# Autodesk Inventor assembly: P1704_E2
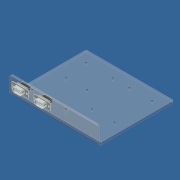
[picture p0: Inventor's stored thumbnail of the model, 180x180]
Saved by Autodesk Inventor 2015 SP2 (Build 190223200, 223)
## iProperties
Created: 2018-05-15
Part Number: P1704_E2
Project: Manette arcade
Description: Console
Document SubType Name: Assembly
Designer: Alexandre.PICOTTE
Author: Alexandre.PICOTTE
## Documents named in this file (3)
- C:\Users\Alexandre.PICOTTE\Documents\P1704_Manettes\06_Dessins\Manette_arcade\P1704_E2.iam
- C:\Users\Alexandre.PICOTTE\Documents\P1704_Manettes\06_Dessins\Manette_arcade\P1704_007.ipt
- C:\Users\Alexandre.PICOTTE\Documents\Inventor\Content Center Files\R2015\fr-FR\D-Sub Male Crimp\D-Sub Male Crimp 9CKT.ipt
## Components (3 placed, 2 different names)
1. P1704_007:1 — Placage:1, Placage:2, Placage:3, Placage:4, Angle:1, Angle:2
2. Sertissage mâle D-Sub D-Sub Male Crimp 9CKT:1 — Placage:1, Placage:3, Angle:1
3. Sertissage mâle D-Sub D-Sub Male Crimp 9CKT:2 — Placage:2, Placage:4, Angle:2
## Relationships (6: Mate 4, Angle 2)
- Placage:1 [Mate]: P1704_007:1 ↔ Sertissage mâle D-Sub D-Sub Male Crimp 9CKT:1
- Placage:2 [Mate]: P1704_007:1 ↔ Sertissage mâle D-Sub D-Sub Male Crimp 9CKT:2
- Placage:3 [Mate]: P1704_007:1 ↔ Sertissage mâle D-Sub D-Sub Male Crimp 9CKT:1
- Placage:4 [Mate]: P1704_007:1 ↔ Sertissage mâle D-Sub D-Sub Male Crimp 9CKT:2
- Angle:1 (0 deg): P1704_007:1 ↔ Sertissage mâle D-Sub D-Sub Male Crimp 9CKT:1
- Angle:2 (0 deg): P1704_007:1 ↔ Sertissage mâle D-Sub D-Sub Male Crimp 9CKT:2
